# Autodesk Inventor assembly: Full
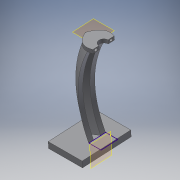
[picture p0: Inventor's stored thumbnail of the model, 180x180]
Saved by Autodesk Inventor 2016 (Build 200138000, 138)
## iProperties
Created: 2018-06-11
Part Number: Full
Document SubType Name: Assembly
Designer: Jorian Bruslind
Author: Jorian Bruslind
## Documents named in this file (4)
- C:\Users\Jorian Bruslind\Documents\GitHub\PersonalProjects\Inventor Projects\Maglev_v2\Full.iam
- C:\Users\Jorian Bruslind\Documents\GitHub\PersonalProjects\Inventor Projects\Maglev_v2\Holder_Side.ipt
- C:\Users\Jorian Bruslind\Documents\GitHub\PersonalProjects\Inventor Projects\Maglev_v2\Stand.ipt
- C:\Users\Jorian Bruslind\Documents\GitHub\PersonalProjects\Inventor Projects\Maglev_v2\Base.ipt
## Components (3 placed, 3 different names)
1. Holder_Side:1 — Mate:1, Mate:2, Flush:1
2. Stand:1 — Mate:1, Mate:2, Mate:3
3. Base:1 — Mate:3, Flush:1
## Relationships (4: Mate 3, Flush 1)
- Mate:1: Holder_Side:1 ↔ Stand:1
- Mate:2 (-6.35 mm): Holder_Side:1 ↔ Stand:1
- Mate:3: Stand:1 ↔ Base:1
- Flush:1: Holder_Side:1 ↔ Base:1
